# Autodesk Inventor assembly: Body2
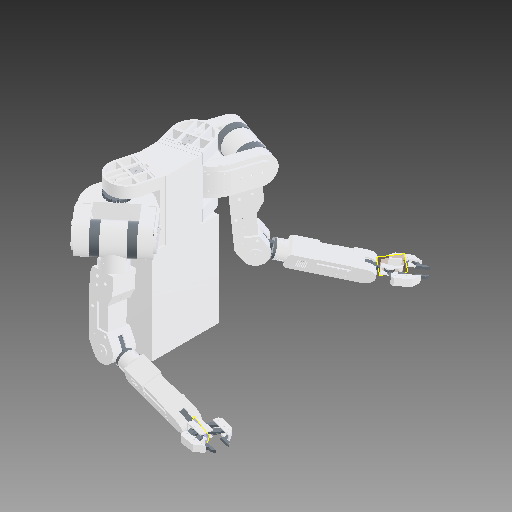
[picture p0: Inventor's stored thumbnail of the model, 512x512]
Saved by Autodesk Inventor 2017 SP1 (Build 210196100, 196)
## iProperties
Created: 2017-06-21
Part Number: Body2
Document SubType Name: Assembly
Designer: zallen
Author: zallen
## Documents named in this file (3)
- C:\Users\Zach\Documents\GitHub\cr-laundry-robot\src\Body 2\Body2.iam
- C:\Users\Zach\Documents\GitHub\cr-laundry-robot\src\Body 2\Torso Assembly\Torso.iam
- C:\Users\Zach\Documents\GitHub\cr-laundry-robot\src\Body\Arm Assembly\ArmAssembly.iam
## Components (3 placed, 2 different names)
1. Torso:1 [sub-assembly] — Mate:1, Mate:2, Mate:3, Mate:4, Mate:5, Mate:6
2. ArmAssembly:1 [sub-assembly] — Mate:1, Mate:2, Mate:3
3. ArmAssembly:2 [sub-assembly] — Mate:4, Mate:5, Mate:6
## Relationships (6: Mate 6)
- Mate:1: Torso:1 ↔ ArmAssembly:1
- Mate:2: Torso:1 ↔ ArmAssembly:1
- Mate:3: Torso:1 ↔ ArmAssembly:1
- Mate:4: Torso:1 ↔ ArmAssembly:2
- Mate:5: Torso:1 ↔ ArmAssembly:2
- Mate:6: Torso:1 ↔ ArmAssembly:2
